# Autodesk Inventor assembly: Assembly1
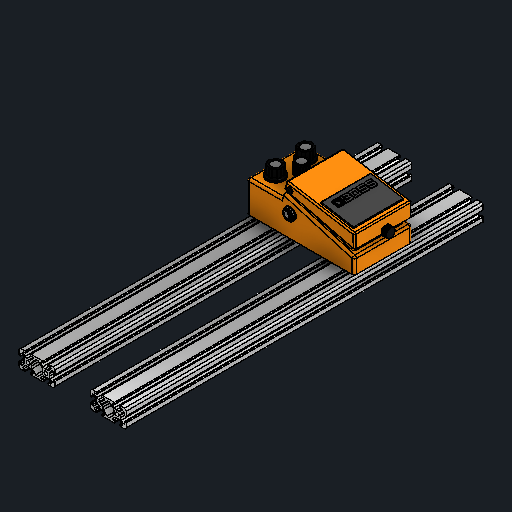
[picture p0: Inventor's stored thumbnail of the model, 512x512]
Saved by Autodesk Inventor 2026.2 (Build 302298000, 298)
## iProperties
Created: 2026-07-17
Part Number: Assembly1
Document SubType Name: Assembly
Designer: JoshuaEah
Author: JoshuaEah
## Documents named in this file (3)
- C:\Users\JoshuaEah\Documents\GitHub\Designed-Trinkets\Guitar\Modular Pedalboard\Assembly1.iam
- C:\Users\JoshuaEah\Documents\GitHub\Designed-Trinkets\Guitar\Modular Pedalboard\2040x40cm Extrusion.ipt
- C:\Users\JoshuaEah\Documents\GitHub\Designed-Trinkets\Guitar\Modular Pedalboard\Pedals\Boss Pedal\Boss_Assembly.iam
## Components (3 placed, 2 different names)
1. 2040x40cm Extrusion:1 — Mate:1, Rigid:1, Mate:2
2. 2040x40cm Extrusion:2 — Rigid:1
3. Boss_Assembly:1 [sub-assembly] — Mate:2
## Relationships (3: Mate 2, WeldJoint 1)
- Mate:1: 2040x40cm Extrusion:1
- Rigid:1 [WeldJoint] (40 mm): 2040x40cm Extrusion:1 ↔ 2040x40cm Extrusion:2
- Mate:2: 2040x40cm Extrusion:1 ↔ Boss_Assembly:1
